# Autodesk Inventor assembly: NathannInventor
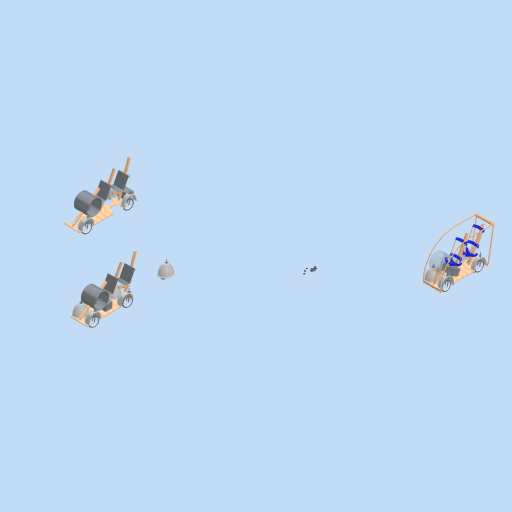
[picture p0: Inventor's stored thumbnail of the model, 512x512]
Saved by Autodesk Inventor 2023 (Build 270158000, 158)
## iProperties
Created: 2026-03-19
Part Number: NathannInventor
Document SubType Name: Assembly
Designer: Nathann
Mass: 293370 g
Surface Area: 199015 cm^2
Volume: 293370 cm^3
Density: 1 g/cm^3
Author: Nathann
## Documents named in this file (23)
- C:\Users\Nathann\ClawdDrive\Objet3D\neodrive\neodrive-cad-ergonomic-v1\NathannCADproposition\NathannInventor.iam
- C:\Users\Nathann\ClawdDrive\Objet3D\neodrive\neodrive-cad-ergonomic-v1\NathannCADproposition\neodrive-cad-ergonomic-v1-AssemblyBattery.ipt
- C:\Users\Nathann\ClawdDrive\Objet3D\neodrive\neodrive-cad-ergonomic-v1\NathannCADproposition\neodrive-cad-ergonomic-v1-AssemblyForkHardpoint001.ipt
- C:\Users\Nathann\ClawdDrive\Objet3D\neodrive\neodrive-cad-ergonomic-v1\NathannCADproposition\neodrive-cad-ergonomic-v1-AssemblylockPlate001.ipt
- C:\Users\Nathann\ClawdDrive\Objet3D\neodrive\neodrive-cad-ergonomic-v1\NathannCADproposition\neodrive-cad-ergonomic-v1-AssemblyPedalDriver.ipt
- C:\Users\Nathann\ClawdDrive\Objet3D\neodrive\neodrive-cad-ergonomic-v1\NathannCADproposition\neodrive-cad-ergonomic-v1-AssemblyRearSeat.ipt
- C:\Users\Nathann\ClawdDrive\Objet3D\neodrive\neodrive-cad-ergonomic-v1\NathannCADproposition\neodrive-cad-ergonomic-v1-AssemblyWheelAndFork005.ipt
- C:\Users\Nathann\ClawdDrive\Objet3D\neodrive\neodrive-cad-ergonomic-v1\eggshellCorePrinted\eggshellCorePrinted.ipt
- C:\Users\Nathann\ClawdDrive\Objet3D\neodrive\neodrive-cad-ergonomic-v1\eggshellCorePrintedLeft.ipt
- C:\Users\Nathann\ClawdDrive\Objet3D\neodrive\neodrive-cad-ergonomic-v1\seat\CurvedSeatHolder.ipt
- C:\Users\Nathann\ClawdDrive\Objet3D\neodrive\neodrive-cad-ergonomic-v1\seat\poutre100x80.ipt
- C:\Users\Nathann\ClawdDrive\Objet3D\neodrive\neodrive-cad-ergonomic-v1\NathannCADproposition\human.ipt
- C:\Users\Nathann\ClawdDrive\Objet3D\neodrive\neodrive-cad-ergonomic-v1\eggshellCorePrinted\rearwheelCorePrintedL.ipt
- C:\Users\Nathann\ClawdDrive\Objet3D\neodrive\neodrive-cad-ergonomic-v1\eggshellCorePrinted\rearwheelCorePrintedR.ipt
- C:\Users\Nathann\ClawdDrive\Objet3D\neodrive\neodrive-cad-ergonomic-v1\NathannCADproposition\SideWoodL.ipt
- C:\Users\Nathann\ClawdDrive\Objet3D\neodrive\neodrive-cad-ergonomic-v1\seat\SeatBeam100x80.ipt
- C:\Users\Nathann\ClawdDrive\Objet3D\neodrive\neodrive-cad-ergonomic-v1\NathannCADproposition\skateboardplank.ipt
- C:\Users\Nathann\ClawdDrive\Objet3D\neodrive\neodrive-cad-ergonomic-v1\NathannCADproposition\mainbeam.ipt
- C:\Users\Nathann\ClawdDrive\Objet3D\neodrive\neodrive-cad-ergonomic-v1\seat\seatButtSidePlate.ipt
- C:\Users\Nathann\ClawdDrive\Objet3D\neodrive\neodrive-cad-ergonomic-v1\seat\SeatBackSidePlate.ipt
- C:\Users\Nathann\ClawdDrive\Objet3D\neodrive\neodrive-cad-ergonomic-v1\NathannCADproposition\lateralReinforcement.ipt
- C:\Users\Nathann\ClawdDrive\Objet3D\neodrive\neodrive-cad-ergonomic-v1\NathannCADproposition\PoutreDirection.ipt
- C:\Users\Nathann\ClawdDrive\Objet3D\neodrive\neodrive-cad-ergonomic-v1\eggshellCorePrinted\hardpoint.iam
## Components (114 placed, 22 different names)
1. neodrive-cad-ergonomic-v1-AssemblyForkHardpoint001:1 — Insert:1, Mate:3, Tangent:1, Tangent:2
2. neodrive-cad-ergonomic-v1-AssemblylockPlate001:1 — Mate:2
3. neodrive-cad-ergonomic-v1-AssemblyPedalDriver:1
4. neodrive-cad-ergonomic-v1-AssemblyRearSeat:1
5. neodrive-cad-ergonomic-v1-AssemblyWheelAndFork005:1 — Mate:2, Insert:1
6. neodrive-cad-ergonomic-v1-AssemblyRearSeat:2
7. eggshellCorePrinted:1 — Flush:1, Mate:3, Tangent:1, Tangent:2, Flush:2, Angle:1, Angle:2, Flush:7
8. eggshellCorePrintedLeft:1 — Tangent:3, Mate:4, Tangent:4, Flush:2, Angle:1, Angle:2, Flush:5
9. neodrive-cad-ergonomic-v1-AssemblyWheelAndFork005:2 — Insert:2
10. neodrive-cad-ergonomic-v1-AssemblyForkHardpoint001:2 — Tangent:3, Mate:4, Tangent:4, Insert:2
11. neodrive-cad-ergonomic-v1-AssemblylockPlate001:2
12. CurvedSeatHolder:1 — Flush:4
13. poutre100x80:1 — Flush:4
14. CurvedSeatHolder:2
15. CurvedSeatHolder:3
16. CurvedSeatHolder:4
17. human:1
18. poutre100x80:2
19. poutre100x80:3 — Mate:5, Flush:6
20. CurvedSeatHolder:5
21. CurvedSeatHolder:6
22. CurvedSeatHolder:7 — Mate:7
23. CurvedSeatHolder:8 — Mate:6
24. neodrive-cad-ergonomic-v1-AssemblyBattery:2
25. neodrive-cad-ergonomic-v1-AssemblyWheelAndFork005:3
26. neodrive-cad-ergonomic-v1-AssemblylockPlate001:3
27. neodrive-cad-ergonomic-v1-AssemblyForkHardpoint001:3
28. rearwheelCorePrintedL:1
29. rearwheelCorePrintedR:1
30. SideWoodL:1 — Flush:5, Flush:44
31. SeatBeam100x80:1
32. SeatBeam100x80:2 — Mate:5, Flush:6, Mate:6, Mate:7
33. skateboardplank:1 — Flush:7
34. skateboardplank:2
35. neodrive-cad-ergonomic-v1-AssemblyForkHardpoint001:5
36. neodrive-cad-ergonomic-v1-AssemblylockPlate001:4
37. neodrive-cad-ergonomic-v1-AssemblyPedalDriver:2
38. neodrive-cad-ergonomic-v1-AssemblyRearSeat:3
39. neodrive-cad-ergonomic-v1-AssemblyWheelAndFork005:5
40. neodrive-cad-ergonomic-v1-AssemblyRearSeat:4
41. eggshellCorePrinted:3
42. eggshellCorePrintedLeft:4
43. neodrive-cad-ergonomic-v1-AssemblyWheelAndFork005:6
44. neodrive-cad-ergonomic-v1-AssemblyForkHardpoint001:6
45. neodrive-cad-ergonomic-v1-AssemblylockPlate001:5
46. CurvedSeatHolder:9
47. poutre100x80:4
48. CurvedSeatHolder:10
49. CurvedSeatHolder:11
50. CurvedSeatHolder:12
51. poutre100x80:5
52. poutre100x80:6
53. CurvedSeatHolder:13
54. CurvedSeatHolder:14
55. CurvedSeatHolder:15
56. CurvedSeatHolder:16
57. neodrive-cad-ergonomic-v1-AssemblyBattery:3
58. neodrive-cad-ergonomic-v1-AssemblyWheelAndFork005:7
59. neodrive-cad-ergonomic-v1-AssemblylockPlate001:6
60. neodrive-cad-ergonomic-v1-AssemblyForkHardpoint001:7
61. SeatBeam100x80:3
62. SeatBeam100x80:4
63. skateboardplank:3
64. skateboardplank:4
65. eggshellCorePrinted:4
66. eggshellCorePrintedLeft:5
67. neodrive-cad-ergonomic-v1-AssemblyForkHardpoint001:8 — Insert:17
68. neodrive-cad-ergonomic-v1-AssemblylockPlate001:7
69. neodrive-cad-ergonomic-v1-AssemblyWheelAndFork005:8
70. eggshellCorePrinted:5 — Flush:18, Flush:19, Mate:21, Insert:17
71. eggshellCorePrintedLeft:6 — Flush:16, Mate:20, Flush:17, Insert:18
72. neodrive-cad-ergonomic-v1-AssemblyWheelAndFork005:9
73. neodrive-cad-ergonomic-v1-AssemblyForkHardpoint001:9 — Insert:18
74. poutre100x80:9 — Mate:26, Mate:27, Mate:28, Mate:29, Flush:34, Flush:35
75. CurvedSeatHolder:21 — Mate:27, Mate:29, Insert:10
76. CurvedSeatHolder:22 — Mate:26, Mate:28, Flush:32, Insert:9, Mate:37
77. CurvedSeatHolder:23 — Mate:31, Flush:28, Flush:29, Flush:30, Mate:33, Mate:34, Mate:35, Flush:31, Flush:33
78. CurvedSeatHolder:24 — Mate:30, Mate:36
79. neodrive-cad-ergonomic-v1-AssemblyBattery:4
80. SeatBeam100x80:6 — Mate:30, Mate:31, Flush:33
81. skateboardplank:5 — Flush:18, Flush:19, Mate:21, Flush:22, Flush:23, Mate:23, Flush:24, Mate:24, Flush:26, Mate:32, Flush:43
82. skateboardplank:6 — Flush:16, Mate:20, Flush:17, Mate:22, Flush:20, Flush:21, Flush:24, Mate:24, Mate:25, Flush:27, Flush:44
83. rearwheelCorePrintedL:2 — Mate:22, Flush:20, Flush:21, Insert:11
84. rearwheelCorePrintedR:2 — Flush:22, Flush:23, Mate:23, Insert:12
85. mainbeam:1 — Flush:26, Mate:32, Flush:27, Flush:34, Flush:35
86. seatButtSidePlate:1 — Flush:28, Mate:35, Flush:31
87. seatButtSidePlate:2 — Flush:29, Flush:30, Mate:33, Mate:34, Mate:36
88. SeatBackSidePlate:1 — Flush:32, Mate:37
89. SeatBackSidePlate:2 — Insert:9, Insert:10
90. neodrive-cad-ergonomic-v1-AssemblyWheelAndFork005:10 — Insert:13
91. neodrive-cad-ergonomic-v1-AssemblyWheelAndFork005:11 — Insert:14
92. neodrive-cad-ergonomic-v1-AssemblyForkHardpoint001:10 — Insert:11, Insert:13
93. neodrive-cad-ergonomic-v1-AssemblyForkHardpoint001:11 — Insert:12, Insert:14
94. poutre100x80:10
95. CurvedSeatHolder:25
96. CurvedSeatHolder:26
97. CurvedSeatHolder:27
98. CurvedSeatHolder:28
99. SeatBeam100x80:7
100. seatButtSidePlate:3
101. seatButtSidePlate:4
102. SeatBackSidePlate:3
103. SeatBackSidePlate:4
104. lateralReinforcement:1 — Flush:43
105. lateralReinforcement:2
106. lateralReinforcement:3 — Mate:52
107. lateralReinforcement:4
108. neodrive-cad-ergonomic-v1-AssemblylockPlate001:8
109. neodrive-cad-ergonomic-v1-AssemblyPedalDriver:3
110. PoutreDirection:1
111. SideWoodL:2 — Mate:52
112. lateralReinforcement:5
113. lateralReinforcement:6
114. hardpoint:1 [sub-assembly]
## Relationships (120: Mate 49, Flush 41, Insert 16, Tangent 8, Angle 6)
- Mate:2: neodrive-cad-ergonomic-v1-AssemblylockPlate001:1 ↔ neodrive-cad-ergonomic-v1-AssemblyWheelAndFork005:1
- Insert:1 (20 mm): neodrive-cad-ergonomic-v1-AssemblyForkHardpoint001:1 ↔ neodrive-cad-ergonomic-v1-AssemblyWheelAndFork005:1
- Flush:1: eggshellCorePrinted:1
- Mate:3: neodrive-cad-ergonomic-v1-AssemblyForkHardpoint001:1 ↔ eggshellCorePrinted:1
- Tangent:1 (5 mm): neodrive-cad-ergonomic-v1-AssemblyForkHardpoint001:1 ↔ eggshellCorePrinted:1
- Tangent:2 (5 mm): neodrive-cad-ergonomic-v1-AssemblyForkHardpoint001:1 ↔ eggshellCorePrinted:1
- Tangent:3 (5 mm): eggshellCorePrintedLeft:1 ↔ neodrive-cad-ergonomic-v1-AssemblyForkHardpoint001:2
- Mate:4: eggshellCorePrintedLeft:1 ↔ neodrive-cad-ergonomic-v1-AssemblyForkHardpoint001:2
- Tangent:4 (5 mm): eggshellCorePrintedLeft:1 ↔ neodrive-cad-ergonomic-v1-AssemblyForkHardpoint001:2
- Flush:2: eggshellCorePrinted:1 ↔ eggshellCorePrintedLeft:1
- Insert:2 (20 mm): neodrive-cad-ergonomic-v1-AssemblyWheelAndFork005:2 ↔ neodrive-cad-ergonomic-v1-AssemblyForkHardpoint001:2
- Angle:1 (180 deg): eggshellCorePrinted:1 ↔ eggshellCorePrintedLeft:1
- Angle:2 (0 deg): eggshellCorePrinted:1 ↔ eggshellCorePrintedLeft:1
- Flush:4 (-700 mm): CurvedSeatHolder:1 ↔ poutre100x80:1
- Flush:5: eggshellCorePrintedLeft:1 ↔ SideWoodL:1
- Mate:5: poutre100x80:3 ↔ SeatBeam100x80:2
- Flush:6: poutre100x80:3 ↔ SeatBeam100x80:2
- Mate:6: CurvedSeatHolder:8 ↔ SeatBeam100x80:2
- Mate:7: CurvedSeatHolder:7 ↔ SeatBeam100x80:2
- Flush:7: eggshellCorePrinted:1 ↔ skateboardplank:1
- [Mate]: neodrive-cad-ergonomic-v1-AssemblylockPlate001:4 ↔ neodrive-cad-ergonomic-v1-AssemblyWheelAndFork005:5
- [Insert] (20 mm): neodrive-cad-ergonomic-v1-AssemblyForkHardpoint001:5 ↔ neodrive-cad-ergonomic-v1-AssemblyWheelAndFork005:5
- [Mate]: neodrive-cad-ergonomic-v1-AssemblyForkHardpoint001:5 ↔ eggshellCorePrinted:3
- [Tangent] (5 mm): neodrive-cad-ergonomic-v1-AssemblyForkHardpoint001:5 ↔ eggshellCorePrinted:3
- [Tangent] (5 mm): neodrive-cad-ergonomic-v1-AssemblyForkHardpoint001:5 ↔ eggshellCorePrinted:3
- [Tangent] (5 mm): eggshellCorePrintedLeft:4 ↔ neodrive-cad-ergonomic-v1-AssemblyForkHardpoint001:6
- [Mate]: eggshellCorePrintedLeft:4 ↔ neodrive-cad-ergonomic-v1-AssemblyForkHardpoint001:6
- [Tangent] (5 mm): eggshellCorePrintedLeft:4 ↔ neodrive-cad-ergonomic-v1-AssemblyForkHardpoint001:6
- [Flush]: eggshellCorePrinted:3 ↔ eggshellCorePrintedLeft:4
- [Insert] (20 mm): neodrive-cad-ergonomic-v1-AssemblyWheelAndFork005:6 ↔ neodrive-cad-ergonomic-v1-AssemblyForkHardpoint001:6
- [Angle] (180 deg): eggshellCorePrinted:3 ↔ eggshellCorePrintedLeft:4
- [Angle] (0 deg): eggshellCorePrinted:3 ↔ eggshellCorePrintedLeft:4
- [Flush] (-700 mm): CurvedSeatHolder:9 ↔ poutre100x80:4
- [Mate]: poutre100x80:6 ↔ SeatBeam100x80:4
- [Flush]: poutre100x80:6 ↔ SeatBeam100x80:4
- [Mate]: CurvedSeatHolder:16 ↔ SeatBeam100x80:4
- [Mate]: CurvedSeatHolder:15 ↔ SeatBeam100x80:4
- [Flush]: eggshellCorePrinted:3 ↔ skateboardplank:3
- [Mate]: neodrive-cad-ergonomic-v1-AssemblylockPlate001:7 ↔ neodrive-cad-ergonomic-v1-AssemblyWheelAndFork005:8
- [Insert] (20 mm): neodrive-cad-ergonomic-v1-AssemblyForkHardpoint001:8 ↔ neodrive-cad-ergonomic-v1-AssemblyWheelAndFork005:8
- [Flush]: eggshellCorePrinted:5 ↔ eggshellCorePrintedLeft:6
- [Insert] (20 mm): neodrive-cad-ergonomic-v1-AssemblyWheelAndFork005:9 ↔ neodrive-cad-ergonomic-v1-AssemblyForkHardpoint001:9
- [Angle] (180 deg): eggshellCorePrinted:5 ↔ eggshellCorePrintedLeft:6
- [Angle] (0 deg): eggshellCorePrinted:5 ↔ eggshellCorePrintedLeft:6
- [Mate]: poutre100x80:9 ↔ SeatBeam100x80:6
- [Flush]: poutre100x80:9 ↔ SeatBeam100x80:6
- [Mate]: CurvedSeatHolder:24 ↔ SeatBeam100x80:6
- [Mate]: CurvedSeatHolder:23 ↔ SeatBeam100x80:6
- [Flush]: eggshellCorePrinted:5 ↔ skateboardplank:5
- Flush:16: eggshellCorePrintedLeft:6 ↔ skateboardplank:6
- Mate:20: eggshellCorePrintedLeft:6 ↔ skateboardplank:6
- Flush:17: eggshellCorePrintedLeft:6 ↔ skateboardplank:6
- Flush:18: eggshellCorePrinted:5 ↔ skateboardplank:5
- Flush:19: eggshellCorePrinted:5 ↔ skateboardplank:5
- Mate:21: eggshellCorePrinted:5 ↔ skateboardplank:5
- Mate:22: skateboardplank:6 ↔ rearwheelCorePrintedL:2
- Flush:20: skateboardplank:6 ↔ rearwheelCorePrintedL:2
- Flush:21: skateboardplank:6 ↔ rearwheelCorePrintedL:2
- Flush:22: skateboardplank:5 ↔ rearwheelCorePrintedR:2
- Flush:23: skateboardplank:5 ↔ rearwheelCorePrintedR:2
- Mate:23: skateboardplank:5 ↔ rearwheelCorePrintedR:2
- Flush:24: skateboardplank:5 ↔ skateboardplank:6
- Mate:24: skateboardplank:5 ↔ skateboardplank:6
- Mate:25: skateboardplank:6
- Mate:26: poutre100x80:9 ↔ CurvedSeatHolder:22
- Mate:27: poutre100x80:9 ↔ CurvedSeatHolder:21
- Mate:28: poutre100x80:9 ↔ CurvedSeatHolder:22
- Mate:29: poutre100x80:9 ↔ CurvedSeatHolder:21
- Mate:30: CurvedSeatHolder:24 ↔ SeatBeam100x80:6
- Mate:31: CurvedSeatHolder:23 ↔ SeatBeam100x80:6
- Flush:26: skateboardplank:5 ↔ mainbeam:1
- Mate:32: skateboardplank:5 ↔ mainbeam:1
- Flush:27 (410 mm): skateboardplank:6 ↔ mainbeam:1
- Flush:28: CurvedSeatHolder:23 ↔ seatButtSidePlate:1
- Flush:29: CurvedSeatHolder:23 ↔ seatButtSidePlate:2
- Flush:30: CurvedSeatHolder:23 ↔ seatButtSidePlate:2
- Mate:33: CurvedSeatHolder:23 ↔ seatButtSidePlate:2
- Mate:34: CurvedSeatHolder:23 ↔ seatButtSidePlate:2
- Mate:35: CurvedSeatHolder:23 ↔ seatButtSidePlate:1
- Flush:31: CurvedSeatHolder:23 ↔ seatButtSidePlate:1
- Mate:36: CurvedSeatHolder:24 ↔ seatButtSidePlate:2
- Flush:32: CurvedSeatHolder:22 ↔ SeatBackSidePlate:1
- Insert:9: CurvedSeatHolder:22 ↔ SeatBackSidePlate:2
- Insert:10: CurvedSeatHolder:21 ↔ SeatBackSidePlate:2
- Mate:37: CurvedSeatHolder:22 ↔ SeatBackSidePlate:1
- Flush:33: CurvedSeatHolder:23 ↔ SeatBeam100x80:6
- Insert:11: rearwheelCorePrintedL:2 ↔ neodrive-cad-ergonomic-v1-AssemblyForkHardpoint001:10
- Insert:12: rearwheelCorePrintedR:2 ↔ neodrive-cad-ergonomic-v1-AssemblyForkHardpoint001:11
- Insert:13: neodrive-cad-ergonomic-v1-AssemblyWheelAndFork005:10 ↔ neodrive-cad-ergonomic-v1-AssemblyForkHardpoint001:10
- Insert:14: neodrive-cad-ergonomic-v1-AssemblyWheelAndFork005:11 ↔ neodrive-cad-ergonomic-v1-AssemblyForkHardpoint001:11
- Flush:34: poutre100x80:9 ↔ mainbeam:1
- Flush:35 (35 mm): poutre100x80:9 ↔ mainbeam:1
- [Mate]: poutre100x80:10 ↔ SeatBeam100x80:7
- [Flush]: poutre100x80:10 ↔ SeatBeam100x80:7
- [Mate]: CurvedSeatHolder:28 ↔ SeatBeam100x80:7
- [Mate]: CurvedSeatHolder:27 ↔ SeatBeam100x80:7
- [Mate]: poutre100x80:10 ↔ CurvedSeatHolder:26
- [Mate]: poutre100x80:10 ↔ CurvedSeatHolder:25
- [Mate]: poutre100x80:10 ↔ CurvedSeatHolder:26
- [Mate]: poutre100x80:10 ↔ CurvedSeatHolder:25
- [Mate]: CurvedSeatHolder:28 ↔ SeatBeam100x80:7
- [Mate]: CurvedSeatHolder:27 ↔ SeatBeam100x80:7
- [Flush]: CurvedSeatHolder:27 ↔ seatButtSidePlate:3
- [Flush]: CurvedSeatHolder:27 ↔ seatButtSidePlate:4
- [Flush]: CurvedSeatHolder:27 ↔ seatButtSidePlate:4
- [Mate]: CurvedSeatHolder:27 ↔ seatButtSidePlate:4
- [Mate]: CurvedSeatHolder:27 ↔ seatButtSidePlate:4
- [Mate]: CurvedSeatHolder:27 ↔ seatButtSidePlate:3
- [Flush]: CurvedSeatHolder:27 ↔ seatButtSidePlate:3
- [Mate]: CurvedSeatHolder:28 ↔ seatButtSidePlate:4
- [Flush]: CurvedSeatHolder:26 ↔ SeatBackSidePlate:3
- [Insert]: CurvedSeatHolder:26 ↔ SeatBackSidePlate:4
- [Insert]: CurvedSeatHolder:25 ↔ SeatBackSidePlate:4
- [Mate]: CurvedSeatHolder:26 ↔ SeatBackSidePlate:3
- [Flush]: CurvedSeatHolder:27 ↔ SeatBeam100x80:7
- Insert:17: neodrive-cad-ergonomic-v1-AssemblyForkHardpoint001:8 ↔ eggshellCorePrinted:5
- Insert:18: eggshellCorePrintedLeft:6 ↔ neodrive-cad-ergonomic-v1-AssemblyForkHardpoint001:9
- Flush:43: skateboardplank:5 ↔ lateralReinforcement:1
- Flush:44: SideWoodL:1 ↔ skateboardplank:6
- Mate:52: lateralReinforcement:3 ↔ SideWoodL:2
## Named parameters: d33_d25 = 0 mm, d34_d26 = 0 mm, d35_d9 = 0 mm, d36_d10 = 5 mm, d37_d11 = 5 mm, d38_d12 = 5 mm, d39_d13 = 0 mm, d40_d14 = 5 mm, d41_d15 = 0 mm, d42_d16 = 20 mm, d43_d17 = 180 deg, d44_d18 = 0 deg, d45_d20 = -700 mm, d46_d22 = 0 mm, d47_d23 = 0 mm, d48_d24 = 0 mm, d49_d1 = 0 mm, d50_d3 = 20 mm, d51_d33_d25 = 0 mm, d52_d34_d26 = 0 mm, d59_d41_d15 = 0 mm, d60_d42_d16 = 20 mm, d61_d43_d17 = 180 deg, d62_d44_d18 = 0 deg, d64_d46_d22 = 0 mm, d65_d47_d23 = 0 mm, d66_d48_d24 = 0 mm, d67_d49_d1 = 0 mm, d68_d50_d3 = 20 mm, d116_d98 = 0 mm, d117_d99 = 0 mm, d118_d100 = 0 mm, d119_d101 = 0 mm, d120_d102 = 0 mm, d121_d103 = 0 mm, d122_d104 = 0 mm, d123_d105 = 0 mm, d124_d106 = 0 mm, d125_d107 = 0 mm, d126_d108 = 0 mm, d127_d109 = 0 mm, d128_d51_d33_d25 = 0 mm, d129_d64_d46_d22 = 0 mm, d130_d65_d47_d23 = 0 mm, d131_d66_d48_d24 = 0 mm, d132_d85 = 0 mm, d133_d86 = 0 mm, d134_d87 = 0 mm, d135_d88 = 0 mm, d136_d89 = 0 mm, d137_d90 = 0 mm, d138_d94 = 0 mm
